# Autodesk Inventor assembly: test
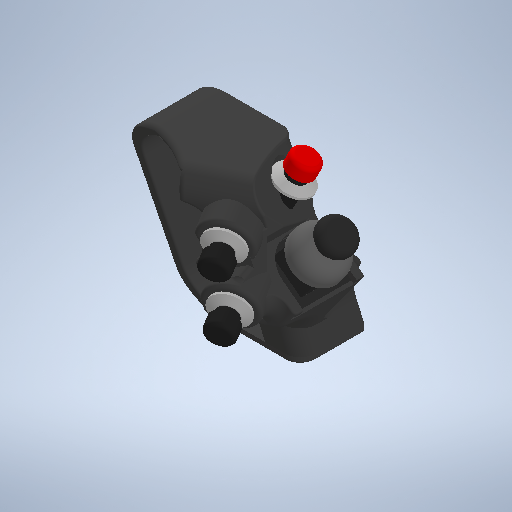
[picture p0: Inventor's stored thumbnail of the model, 512x512]
Saved by Autodesk Inventor 2026.1 (Build 301233020, 233B)
## iProperties
Created: 2026-01-20
Part Number: test
Document SubType Name: Assembly
Designer: hibik
Author: hibik
## Documents named in this file (5)
- C:\Users\hibik\Documents\Robomech\HR\controller\test.iam
- C:\Users\hibik\Documents\Robomech\HR\controller\base.ipt
- C:\Users\hibik\Documents\Robomech\HR\controller\pannel_push_sw.ipt
- C:\Users\hibik\Documents\Robomech\HR\controller\stick.ipt
- C:\Users\hibik\Documents\Robomech\HR\controller\pannel_push_sw._red.ipt
## Components (5 placed, 4 different names)
1. base:1 — メイト:3, メイト:4, メイト:5, 挿入:1, 挿入:2, 挿入:3
2. pannel_push_sw:1 — 挿入:1
3. pannel_push_sw:2 — 挿入:2
4. stick:1 — メイト:3, メイト:4, メイト:5
5. pannel_push_sw._red:1 — 挿入:3
## Relationships (6: Mate 3, Insert 3)
- メイト:3 [Mate]: base:1 ↔ stick:1
- メイト:4 [Mate] (0.5 mm): base:1 ↔ stick:1
- メイト:5 [Mate] (0.5 mm): base:1 ↔ stick:1
- 挿入:1 [Insert]: base:1 ↔ pannel_push_sw:1
- 挿入:2 [Insert]: base:1 ↔ pannel_push_sw:2
- 挿入:3 [Insert]: base:1 ↔ pannel_push_sw._red:1
